# Autodesk Inventor assembly: ManzanaD68mm
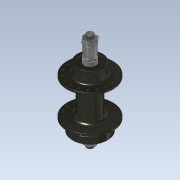
[picture p0: Inventor's stored thumbnail of the model, 180x180]
Saved by Autodesk Inventor 2021 (Build 250183000, 183)
## iProperties
Created: 2016-06-28
Part Number: ManzanaD68mm
Document SubType Name: Assembly
Designer: YeseF
Mass: 375.635 g
Surface Area: 453.176 cm^2
Volume: 107.624 cm^3
Density: 3.49025 g/cm^3
Author: YeseF
## Documents named in this file (8)
- G:\Unidades compartidas\APM\02 Inventor-Drive\ManzanaT68mm\ManzanaT68mm.iam
- G:\Unidades compartidas\APM\02 Inventor-Drive\ManzanaT68mm\ManzanaT_68mm_disco.ipt
- G:\Unidades compartidas\APM\02 Inventor-Drive\ManzanaT68mm\TuercaT_eje.ipt
- G:\Unidades compartidas\APM\02 Inventor-Drive\ManzanaT68mm\EjeManzanaT.ipt
- G:\Unidades compartidas\APM\02 Inventor-Drive\ManzanaT68mm\TuercaManzana.ipt
- G:\Unidades compartidas\APM\02 Inventor-Drive\ManzanaT68mm\Separador16mm.ipt
- G:\Unidades compartidas\APM\02 Inventor-Drive\ManzanaT68mm\Separador16mm2.ipt
- G:\Unidades compartidas\APM\02 Inventor-Drive\ManzanaT68mm\Separador18mm.ipt
## Components (9 placed, 7 different names)
1. ManzanaT_68mm_disco:1 — Insertar:15, Insertar:16
2. TuercaT_eje:2 — Insert:10, Insertar:16
3. EjeManzanaT:1 — Mate:1, Flush:1, Insertar:14
4. TuercaT_eje:3 — Insert:9, Insertar:15
5. Separador16mm:1 — Insert:10, Insert:11
6. Separador16mm2:1 — Insert:11, Insert:12
7. Separador18mm:1 — Insert:9, Insert:13
8. TuercaManzana:1 — Insert:12
9. TuercaManzana:2 — Insert:13, Flush:1, Insertar:14
## Relationships (10: Insert 8, Mate 1, Flush 1)
- Mate:1: EjeManzanaT:1
- Insert:9: TuercaT_eje:3 ↔ Separador18mm:1
- Insert:10: TuercaT_eje:2 ↔ Separador16mm:1
- Insert:11: Separador16mm:1 ↔ Separador16mm2:1
- Insert:12: Separador16mm2:1 ↔ TuercaManzana:1
- Insert:13: Separador18mm:1 ↔ TuercaManzana:2
- Flush:1 (-5.4 mm): EjeManzanaT:1 ↔ TuercaManzana:2
- Insertar:14 (5.4 mm): EjeManzanaT:1 ↔ TuercaManzana:2
- Insertar:15: ManzanaT_68mm_disco:1 ↔ TuercaT_eje:3
- Insertar:16: ManzanaT_68mm_disco:1 ↔ TuercaT_eje:2
